# Autodesk Inventor assembly: Assembly 3D Cutting
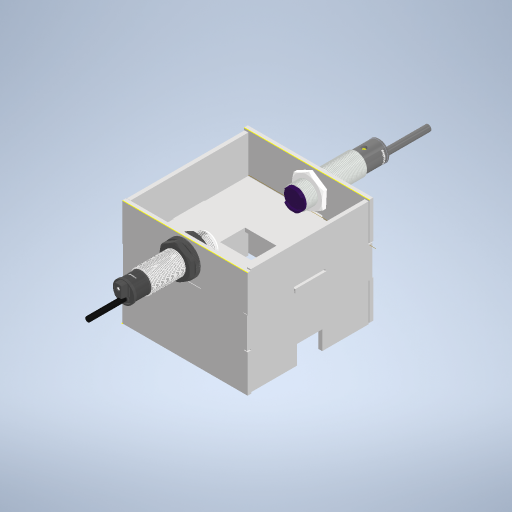
[picture p0: Inventor's stored thumbnail of the model, 512x512]
Saved by Autodesk Inventor 2023 (Build 270158000, 158)
## iProperties
Created: 2023-02-07
Part Number: Assembly 3D Cutting
Document SubType Name: Assembly
Designer: Asus
Author: Asus
## Documents named in this file (6)
- D:\Eksintek\Pneumatik SKUBI Sby\3D Cutting\Assembly 3D Cutting.iam
- D:\Eksintek\Pneumatik SKUBI Sby\3D Cutting\Samping.ipt
- D:\Eksintek\Pneumatik SKUBI Sby\3D Cutting\Depan.ipt
- D:\Eksintek\Pneumatik SKUBI Sby\3D Cutting\bolongan.ipt
- D:\Eksintek\Pneumatik SKUBI Sby\3D Cutting\Library Sensor\BR100-DDT_BR100-DDT-P_BR200-DDTN_BR200-DDTN-P_BR400-DDT_(1)\BR100-DDT_BR100-DDT-P_BR200-DDTN_BR200-DDTN-P_BR400-DDT_(1).ipt
- D:\Eksintek\Pneumatik SKUBI Sby\3D Cutting\Library Sensor\CR18-8DN_CR18-8DP_CR18-8DN2\CR18-8DN_CR18-8DP_CR18-8DN2.ipt
## Components (7 placed, 5 different names)
1. Samping:1
2. Depan:1
3. Depan:2
4. Samping:2 — Mate:2
5. bolongan:1 — Mate:1
6. BR100-DDT_BR100-DDT-P_BR200-DDTN_BR200-DDTN-P_BR400-DDT_(1):1
7. CR18-8DN_CR18-8DP_CR18-8DN2:1
## Relationships (2: Mate 2)
- Mate:1: bolongan:1
- Mate:2: Samping:2
